# Autodesk Inventor assembly: main_pcb.brd
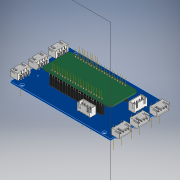
[picture p0: Inventor's stored thumbnail of the model, 180x180]
Saved by Autodesk Inventor 2022 (Build 260153000, 153)
## iProperties
Created: 2021-08-05
Part Number: main_pcb.brd
Document SubType Name: Assembly
Designer: Петров Иван
Mass: 18.6028 g
Surface Area: 275.031 cm^2
Volume: 13.5279 cm^3
Density: 1.37514 g/cm^3
Author: Петров Иван
## Documents named in this file (7)
- C:\Users\Ivan Petrov\Documents\GitHub\OmniBot\design\000.004 - Котроллер СНУ.iam
- C:\Users\Ivan Petrov\Documents\GitHub\OmniBot\design\standart_components\PBS-1.ipt
- C:\Users\Ivan Petrov\Documents\GitHub\OmniBot\design\standart_components\connectrs\JST - XH - Thru (R) - 4Pin - 2.54mm.ipt
- C:\Users\Ivan Petrov\Documents\GitHub\OmniBot\design\000.004.001 - Плата печатная.ipt
- C:\Users\Ivan Petrov\Documents\GitHub\OmniBot\design\standart_components\CONN HEADER VERT 1POS 2.54MM.ipt
- C:\Users\Ivan Petrov\Documents\GitHub\OmniBot\design\standart_components\opencm904.ipt
- C:\Users\Ivan Petrov\Documents\GitHub\OmniBot\design\standart_components\connectrs\JST - XH - Thru (V) - 4Pin - 2.54mm.ipt
## Components (99 placed, 9 different names)
1. 000.004.001 - Плата печатная.ipt:1 — Совмещение:25, Совмещение:26, Совмещение:27, Совмещение:28, Совмещение:29, Совмещение:30, Совмещение:31, Совмещение:32, Совмещение:33, Совмещение:34, Совмещение:35, Совмещение:36, Совмещение:37, Совмещение:38, Совмещение:39, Совмещение:40, Совмещение:41, Совмещение:42, Совмещение:43, Совмещение:44, Совмещение:45, Совмещение:46, Совмещение:47, Совмещение:48, Совмещение:49, Совмещение:50, Совмещение:51, Совмещение:52, Совмещение:53, Совмещение:54, Совмещение:55, Совмещение:56
2. JST - XH - Thru (R) - 4Pin - 2.54mm.ipt:4 — Совмещение:25, Совмещение:26, Совмещение:27
3. opencm904.ipt:1 — Совмещение:23, Совмещение:24, Угол:1
4. JST - XH - Thru (R) - 4Pin - 2.54mm:5 — Совмещение:28, Совмещение:29, Совмещение:30
5. JST - XH - Thru (R) - 4Pin - 2.54mm:6 — Совмещение:31, Совмещение:32, Совмещение:33
6. JST - XH - Thru (R) - 4Pin - 2.54mm:7 — Совмещение:34, Совмещение:35, Совмещение:36
7. JST - XH - Thru (R) - 4Pin - 2.54mm:8 — Совмещение:37, Совмещение:38, Совмещение:39
8. JST - XH - Thru (R) - 4Pin - 2.54mm:9 — Совмещение:40, Совмещение:41, Совмещение:42
9. JST - XH - Thru (V) - 4Pin - 2.54mm:1 — Совмещение:46, Совмещение:47, Совмещение:48
10. JST - XH - Thru (V) - 4Pin - 2.54mm:2 — Совмещение:49, Совмещение:50, Совмещение:51
11. JST - XH - Thru (V) - 4Pin - 2.54mm:3 — Совмещение:54, Совмещение:55, Совмещение:56
12. CONN HEADER VERT 1POS 2.54MM.ipt:1 — Совмещение:21, Совмещение:22, Заподлицо:1, Совмещение:23, Совмещение:24, Угол:1, Совмещение:43
13. PBS-1.ipt:1 — Совмещение:21, Совмещение:22, Заподлицо:1, Угол:2
14. CONN HEADER VERT 1POS 2.54MM:2 — Совмещение:44
15. PBS-1:3
16. CONN HEADER VERT 1POS 2.54MM:3
17. PBS-1:4
18. CONN HEADER VERT 1POS 2.54MM:4
19. PBS-1:5
20. CONN HEADER VERT 1POS 2.54MM:5
21. PBS-1:6
22. CONN HEADER VERT 1POS 2.54MM:6
23. PBS-1:7
24. CONN HEADER VERT 1POS 2.54MM:7
25. PBS-1:8
26. CONN HEADER VERT 1POS 2.54MM:8
27. PBS-1:9
28. CONN HEADER VERT 1POS 2.54MM:9
29. PBS-1:10
30. CONN HEADER VERT 1POS 2.54MM:10
31. PBS-1:11
32. CONN HEADER VERT 1POS 2.54MM:11
33. PBS-1:12
34. CONN HEADER VERT 1POS 2.54MM:12
35. PBS-1:13
36. CONN HEADER VERT 1POS 2.54MM:13
37. PBS-1:14
38. CONN HEADER VERT 1POS 2.54MM:14
39. PBS-1:15
40. CONN HEADER VERT 1POS 2.54MM:15
41. PBS-1:16
42. CONN HEADER VERT 1POS 2.54MM:16
43. PBS-1:17
44. CONN HEADER VERT 1POS 2.54MM:17
45. PBS-1:18
46. CONN HEADER VERT 1POS 2.54MM:18
47. PBS-1:19
48. CONN HEADER VERT 1POS 2.54MM:19
49. PBS-1:20
50. CONN HEADER VERT 1POS 2.54MM:20
51. PBS-1:21
52. CONN HEADER VERT 1POS 2.54MM:21
53. PBS-1:22
54. CONN HEADER VERT 1POS 2.54MM:22
55. PBS-1:23
56. CONN HEADER VERT 1POS 2.54MM:23
57. PBS-1:24
58. CONN HEADER VERT 1POS 2.54MM:24
59. PBS-1:25
60. CONN HEADER VERT 1POS 2.54MM:25
61. PBS-1:26
62. CONN HEADER VERT 1POS 2.54MM:26
63. PBS-1:27
64. CONN HEADER VERT 1POS 2.54MM:27
65. PBS-1:28
66. CONN HEADER VERT 1POS 2.54MM:28
67. PBS-1:29
68. CONN HEADER VERT 1POS 2.54MM:29
69. PBS-1:30
70. CONN HEADER VERT 1POS 2.54MM:30
71. PBS-1:31
72. CONN HEADER VERT 1POS 2.54MM:31
73. PBS-1:32
74. CONN HEADER VERT 1POS 2.54MM:32
75. PBS-1:33
76. CONN HEADER VERT 1POS 2.54MM:33
77. PBS-1:34
78. CONN HEADER VERT 1POS 2.54MM:34
79. PBS-1:35
80. CONN HEADER VERT 1POS 2.54MM:35
81. PBS-1:36
82. CONN HEADER VERT 1POS 2.54MM:36
83. PBS-1:37
84. CONN HEADER VERT 1POS 2.54MM:37
85. PBS-1:38
86. CONN HEADER VERT 1POS 2.54MM:38
87. PBS-1:39
88. CONN HEADER VERT 1POS 2.54MM:39
89. PBS-1:40
90. CONN HEADER VERT 1POS 2.54MM:40
91. PBS-1:41 — Совмещение:45
92. CONN HEADER VERT 1POS 2.54MM:41 — Совмещение:52, Совмещение:53, Угол:2
93. CONN HEADER VERT 1POS 2.54MM:42
94. CONN HEADER VERT 1POS 2.54MM:43
95. CONN HEADER VERT 1POS 2.54MM:44
96. CONN HEADER VERT 1POS 2.54MM:45
97. CONN HEADER VERT 1POS 2.54MM:46
98. CONN HEADER VERT 1POS 2.54MM:47
99. CONN HEADER VERT 1POS 2.54MM:48
## Component patterns: (40 elements, first: CONN HEADER VERT 1POS 2.54MM.ipt:1 + PBS-1.ipt:1), (8 elements, first: CONN HEADER VERT 1POS 2.54MM:41)
## Relationships (39: Mate 36, Angle 2, Flush 1)
- Совмещение:21 [Mate]: CONN HEADER VERT 1POS 2.54MM.ipt:1 ↔ PBS-1.ipt:1
- Совмещение:22 [Mate]: CONN HEADER VERT 1POS 2.54MM.ipt:1 ↔ PBS-1.ipt:1
- Заподлицо:1 [Flush]: CONN HEADER VERT 1POS 2.54MM.ipt:1 ↔ PBS-1.ipt:1
- Совмещение:23 [Mate]: opencm904.ipt:1 ↔ CONN HEADER VERT 1POS 2.54MM.ipt:1
- Совмещение:24 [Mate]: opencm904.ipt:1 ↔ CONN HEADER VERT 1POS 2.54MM.ipt:1
- Совмещение:25 [Mate]: 000.004.001 - Плата печатная.ipt:1 ↔ JST - XH - Thru (R) - 4Pin - 2.54mm.ipt:4
- Совмещение:26 [Mate]: 000.004.001 - Плата печатная.ipt:1 ↔ JST - XH - Thru (R) - 4Pin - 2.54mm.ipt:4
- Совмещение:27 [Mate]: 000.004.001 - Плата печатная.ipt:1 ↔ JST - XH - Thru (R) - 4Pin - 2.54mm.ipt:4
- Совмещение:28 [Mate]: 000.004.001 - Плата печатная.ipt:1 ↔ JST - XH - Thru (R) - 4Pin - 2.54mm:5
- Совмещение:29 [Mate]: 000.004.001 - Плата печатная.ipt:1 ↔ JST - XH - Thru (R) - 4Pin - 2.54mm:5
- Совмещение:30 [Mate]: 000.004.001 - Плата печатная.ipt:1 ↔ JST - XH - Thru (R) - 4Pin - 2.54mm:5
- Совмещение:31 [Mate]: 000.004.001 - Плата печатная.ipt:1 ↔ JST - XH - Thru (R) - 4Pin - 2.54mm:6
- Совмещение:32 [Mate]: 000.004.001 - Плата печатная.ipt:1 ↔ JST - XH - Thru (R) - 4Pin - 2.54mm:6
- Совмещение:33 [Mate]: 000.004.001 - Плата печатная.ipt:1 ↔ JST - XH - Thru (R) - 4Pin - 2.54mm:6
- Совмещение:34 [Mate]: 000.004.001 - Плата печатная.ipt:1 ↔ JST - XH - Thru (R) - 4Pin - 2.54mm:7
- Совмещение:35 [Mate]: 000.004.001 - Плата печатная.ipt:1 ↔ JST - XH - Thru (R) - 4Pin - 2.54mm:7
- Совмещение:36 [Mate]: 000.004.001 - Плата печатная.ipt:1 ↔ JST - XH - Thru (R) - 4Pin - 2.54mm:7
- Совмещение:37 [Mate]: 000.004.001 - Плата печатная.ipt:1 ↔ JST - XH - Thru (R) - 4Pin - 2.54mm:8
- Совмещение:38 [Mate]: 000.004.001 - Плата печатная.ipt:1 ↔ JST - XH - Thru (R) - 4Pin - 2.54mm:8
- Совмещение:39 [Mate]: 000.004.001 - Плата печатная.ipt:1 ↔ JST - XH - Thru (R) - 4Pin - 2.54mm:8
- Совмещение:40 [Mate]: 000.004.001 - Плата печатная.ipt:1 ↔ JST - XH - Thru (R) - 4Pin - 2.54mm:9
- Совмещение:41 [Mate]: 000.004.001 - Плата печатная.ipt:1 ↔ JST - XH - Thru (R) - 4Pin - 2.54mm:9
- Совмещение:42 [Mate]: 000.004.001 - Плата печатная.ipt:1 ↔ JST - XH - Thru (R) - 4Pin - 2.54mm:9
- Угол:1 [Angle] (0 deg): opencm904.ipt:1 ↔ CONN HEADER VERT 1POS 2.54MM.ipt:1
- Совмещение:43 [Mate]: 000.004.001 - Плата печатная.ipt:1 ↔ CONN HEADER VERT 1POS 2.54MM.ipt:1
- Совмещение:44 [Mate]: 000.004.001 - Плата печатная.ipt:1 ↔ CONN HEADER VERT 1POS 2.54MM:2
- Совмещение:45 [Mate]: 000.004.001 - Плата печатная.ipt:1 ↔ PBS-1:41
- Совмещение:46 [Mate]: 000.004.001 - Плата печатная.ipt:1 ↔ JST - XH - Thru (V) - 4Pin - 2.54mm:1
- Совмещение:47 [Mate]: 000.004.001 - Плата печатная.ipt:1 ↔ JST - XH - Thru (V) - 4Pin - 2.54mm:1
- Совмещение:48 [Mate]: 000.004.001 - Плата печатная.ipt:1 ↔ JST - XH - Thru (V) - 4Pin - 2.54mm:1
- Совмещение:49 [Mate]: 000.004.001 - Плата печатная.ipt:1 ↔ JST - XH - Thru (V) - 4Pin - 2.54mm:2
- Совмещение:50 [Mate]: 000.004.001 - Плата печатная.ipt:1 ↔ JST - XH - Thru (V) - 4Pin - 2.54mm:2
- Совмещение:51 [Mate]: 000.004.001 - Плата печатная.ipt:1 ↔ JST - XH - Thru (V) - 4Pin - 2.54mm:2
- Совмещение:52 [Mate]: 000.004.001 - Плата печатная.ipt:1 ↔ CONN HEADER VERT 1POS 2.54MM:41
- Совмещение:53 [Mate]: 000.004.001 - Плата печатная.ipt:1 ↔ CONN HEADER VERT 1POS 2.54MM:41
- Угол:2 [Angle] (0 deg): PBS-1.ipt:1 ↔ CONN HEADER VERT 1POS 2.54MM:41
- Совмещение:54 [Mate]: 000.004.001 - Плата печатная.ipt:1 ↔ JST - XH - Thru (V) - 4Pin - 2.54mm:3
- Совмещение:55 [Mate]: 000.004.001 - Плата печатная.ipt:1 ↔ JST - XH - Thru (V) - 4Pin - 2.54mm:3
- Совмещение:56 [Mate]: 000.004.001 - Плата печатная.ipt:1 ↔ JST - XH - Thru (V) - 4Pin - 2.54mm:3
